# Autodesk Inventor assembly: СБ_Монтажный лист
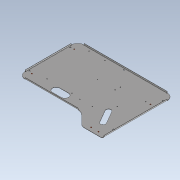
[picture p0: Inventor's stored thumbnail of the model, 180x180]
Saved by Autodesk Inventor 2021.2 (Build 252289000, 289)
## iProperties
Created: 2022-12-06
Part Number: СБ_Монтажный лист
Document SubType Name: Assembly
Designer: Voodoo
Mass: 100.48 g
Surface Area: 1980.5 cm^2
Volume: 98.1157 cm^3
Density: 1.0241 g/cm^3
Author: Voodoo
## Documents named in this file (3)
- C:\Users\Voodoo\Documents\Inventor\АБТ_Инфотабло\СБ_Монтажный лист.iam
- C:\Users\Voodoo\Documents\Inventor\АБТ_Инфотабло\Монтажный лист.ipt
- C:\Users\Voodoo\Documents\Inventor\Content Center Files\R2021\Metizi\Shp_3x8.ipt
## Components (6 placed, 2 different names)
1. Монтажный лист:1 — Вставка:4, Вставка:5
2. Shp_3x8:1
3. Shp_3x8:2
4. Shp_3x8:3 — Вставка:5
5. Shp_3x8:4 — Вставка:4
6. Shp_3x8:5
## Relationships (5: Insert 5)
- [Insert]: Монтажный лист:1 ↔ Shp_3x8:1
- [Insert]: Монтажный лист:1 ↔ Shp_3x8:2
- [Insert]: Монтажный лист:1 ↔ Shp_3x8:5
- Вставка:4 [Insert]: Монтажный лист:1 ↔ Shp_3x8:4
- Вставка:5 [Insert]: Монтажный лист:1 ↔ Shp_3x8:3
